# Autodesk Inventor assembly: Full Bridge
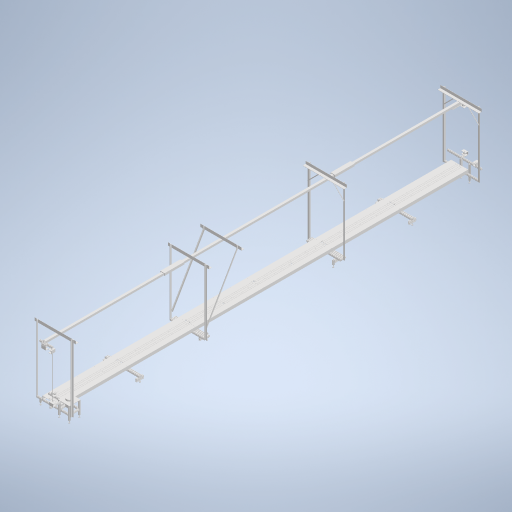
[picture p0: Inventor's stored thumbnail of the model, 512x512]
Saved by Autodesk Inventor 2023 (Build 270158030, 158C)
## iProperties
Created: 2022-07-29
Part Number: Full Bridge
Document SubType Name: Assembly
Designer: jeremyy
Author: jeremyy
## Documents named in this file (6)
- \\andrew.ad.cmu.edu\users\users1\jeremyy\Documents\Inventor\CMU Bridge\New folder\Full Bridge.iam
- \\andrew.ad.cmu.edu\users\users1\jeremyy\Documents\Inventor\CMU Bridge\New folder\Section 2.iam
- \\andrew.ad.cmu.edu\users\users1\jeremyy\Documents\Inventor\CMU Bridge\New folder\Section 3.iam
- \\andrew.ad.cmu.edu\users\users1\jeremyy\Documents\Inventor\CMU Bridge\New folder\Section 1.iam
- \\andrew.ad.cmu.edu\users\users1\jeremyy\Documents\Inventor\CMU Bridge\New folder\LongTop.iam
- \\andrew.ad.cmu.edu\users\users1\jeremyy\Documents\Inventor\CMU Bridge\New folder\VertRod.ipt
## Components (5 placed, 5 different names)
1. Section 2:1 [sub-assembly] — Mate:9, Flush:4, Flush:5, Mate:10, Flush:6, Flush:7
2. Section 3:1 [sub-assembly] — Mate:5, Mate:6, Flush:3, Mate:7, Mate:8, Mate:9, Flush:4, Flush:7
3. Section 1:1 [sub-assembly] — Flush:5, Mate:10, Flush:6
4. LongTop:1 [sub-assembly] — Mate:5, Mate:6, Flush:3
5. VertRod:1 — Mate:7, Mate:8
## Relationships (11: Mate 6, Flush 5)
- Mate:5: Section 3:1 ↔ LongTop:1
- Mate:6 (114.3 mm): Section 3:1 ↔ LongTop:1
- Flush:3 (349.25 mm): Section 3:1 ↔ LongTop:1
- Mate:7: Section 3:1 ↔ VertRod:1
- Mate:8: Section 3:1 ↔ VertRod:1
- Mate:9: Section 2:1 ↔ Section 3:1
- Flush:4: Section 2:1 ↔ Section 3:1
- Flush:5: Section 2:1 ↔ Section 1:1
- Mate:10: Section 2:1 ↔ Section 1:1
- Flush:6: Section 2:1 ↔ Section 1:1
- Flush:7: Section 2:1 ↔ Section 3:1
